# Autodesk Inventor assembly: motherboard_asm
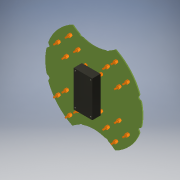
[picture p0: Inventor's stored thumbnail of the model, 180x180]
Saved by Autodesk Inventor 2020 (Build 240168000, 168)
## iProperties
Created: 2024-11-03
Part Number: motherboard_asm
Document SubType Name: Assembly
Designer: Ivan
Author: Ivan
## Documents named in this file (7)
- C:\!projects\DASH_\3D\Dash-V1\motherboard\motherboard_asm.iam
- C:\!projects\DASH_\3D\Dash-V1\motherboard\motherboard.ipt
- C:\!projects\DASH_\3D\Dash-V1\boost.ipt
- C:\!projects\DASH_\3D\Dash-V1\step\m3_bolt\m3x8\Spacer Bolts_m3_bn_L5.ipt
- C:\!projects\DASH_\3D\Dash-V1\step\m3_bolt\Spacer Bolts_m3_bn_L5_ЗЕРКАЛО.ipt
- C:\!projects\DASH_\3D\Dash-V1\step\m3_bolt\Spacer Bolts_m3_bn_L5_ЗЕРКАЛО1.ipt
- C:\!projects\DASH_\3D\Dash-V1\step\m3_bolt\Spacer Bolts_m3_bn_L5_ЗЕРКАЛО_ЗЕРКАЛО.ipt
## Components (22 placed, 6 different names)
1. motherboard:1 — Совмещение:1, Совмещение:2, Угол:1, Вставка:1, Вставка:3, Вставка:4, Вставка:6, Вставка:7, Вставка:8, Вставка:9, Вставка:10
2. Spacer Bolts_m3_bn_L5:4 — Вставка:4, Вставка:5
3. Spacer Bolts_m3_bn_L5:3 — Вставка:6
4. Spacer Bolts_m3_bn_L5:2 — Вставка:1
5. Spacer Bolts_m3_bn_L5:1 — Вставка:3, Совмещение:3
6. boost:1 — Вставка:5, Совмещение:3
7. Spacer Bolts_m3_bn_L5:6 — Вставка:8
8. Spacer Bolts_m3_bn_L5:7 — Вставка:7
9. Spacer Bolts_m3_bn_L5:8 — Вставка:10
10. Spacer Bolts_m3_bn_L5_ЗЕРКАЛО:1
11. Spacer Bolts_m3_bn_L5_ЗЕРКАЛО:2
12. Spacer Bolts_m3_bn_L5_ЗЕРКАЛО:3
13. Spacer Bolts_m3_bn_L5_ЗЕРКАЛО:4
14. Spacer Bolts_m3_bn_L5_ЗЕРКАЛО1:1
15. Spacer Bolts_m3_bn_L5_ЗЕРКАЛО1:2
16. Spacer Bolts_m3_bn_L5_ЗЕРКАЛО1:3
17. Spacer Bolts_m3_bn_L5_ЗЕРКАЛО1:4
18. Spacer Bolts_m3_bn_L5_ЗЕРКАЛО_ЗЕРКАЛО:1
19. Spacer Bolts_m3_bn_L5_ЗЕРКАЛО_ЗЕРКАЛО:2
20. Spacer Bolts_m3_bn_L5_ЗЕРКАЛО_ЗЕРКАЛО:3
21. Spacer Bolts_m3_bn_L5_ЗЕРКАЛО_ЗЕРКАЛО:4
22. Spacer Bolts_m3_bn_L5:5 — Вставка:9
## Relationships (13: Insert 9, Mate 3, Angle 1)
- Совмещение:1 [Mate]: motherboard:1
- Совмещение:2 [Mate]: motherboard:1
- Угол:1 [Angle] (-45 deg): motherboard:1
- Вставка:1 [Insert]: motherboard:1 ↔ Spacer Bolts_m3_bn_L5:2
- Вставка:3 [Insert]: motherboard:1 ↔ Spacer Bolts_m3_bn_L5:1
- Вставка:4 [Insert]: motherboard:1 ↔ Spacer Bolts_m3_bn_L5:4
- Вставка:5 [Insert]: Spacer Bolts_m3_bn_L5:4 ↔ boost:1
- Совмещение:3 [Mate]: Spacer Bolts_m3_bn_L5:1 ↔ boost:1
- Вставка:6 [Insert]: motherboard:1 ↔ Spacer Bolts_m3_bn_L5:3
- Вставка:7 [Insert] (5 mm): motherboard:1 ↔ Spacer Bolts_m3_bn_L5:7
- Вставка:8 [Insert] (5 mm): motherboard:1 ↔ Spacer Bolts_m3_bn_L5:6
- Вставка:9 [Insert] (5 mm): motherboard:1 ↔ Spacer Bolts_m3_bn_L5:5
- Вставка:10 [Insert] (5 mm): motherboard:1 ↔ Spacer Bolts_m3_bn_L5:8
